# Autodesk Inventor assembly: slozene
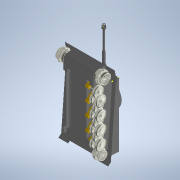
[picture p0: Inventor's stored thumbnail of the model, 180x180]
Saved by Autodesk Inventor 2022 (Build 260153000, 153)
## iProperties
Created: 2022-11-15
Part Number: slozene
Document SubType Name: Assembly
Designer: matys
Author: matys
## Documents named in this file (24)
- C:\Users\matys\Desktop\Práce4tak\Inventor\novy tank\model\slozene.iam
- C:\Users\matys\Desktop\Práce4tak\Inventor\novy tank\model\dolni-cast.ipt
- C:\Users\matys\Desktop\Práce4tak\Inventor\model_v1\motor.ipt
- C:\Users\matys\Desktop\Práce4tak\Inventor\novy tank\ozubene-kolo.ipt
- C:\Users\matys\Desktop\Práce4tak\Inventor\mechanismus_odpruzeni\pist.ipt
- C:\Users\matys\Desktop\Práce4tak\Inventor\mechanismus_odpruzeni\pist-dolni.ipt
- C:\Users\matys\Desktop\Práce4tak\Inventor\mechanismus_odpruzeni\pist-zatka.ipt
- C:\Users\matys\Desktop\Práce4tak\Inventor\mechanismus_odpruzeni\mid.ipt
- C:\Users\matys\Desktop\Práce4tak\Inventor\novy tank\tycinka.ipt
- C:\Users\matys\Desktop\Práce4tak\Inventor\novy tank\tycinka_12mm.ipt
- C:\Users\matys\Desktop\Práce4tak\Inventor\novy tank\spring.ipt
- C:\Users\matys\Desktop\Práce4tak\Inventor\novy tank\tycinka_dlouha.ipt
- C:\Users\matys\Desktop\Práce4tak\Inventor\novy tank\kolo_mensi.ipt
- C:\Users\matys\Desktop\Práce4tak\Inventor\novy tank\sroub.ipt
- C:\Users\matys\Desktop\Práce4tak\Inventor\novy tank\tycinka_kratsi.ipt
- C:\Users\matys\Desktop\Práce4tak\Inventor\novy tank\kolo_vetsi.ipt
- C:\Users\matys\Desktop\Práce4tak\Inventor\novy tank\ozubene-kolo_mini.ipt
- C:\Users\matys\Desktop\Práce4tak\Inventor\baterka.ipt
- C:\Users\matys\Desktop\Práce4tak\Inventor\model_v1\L298N.ipt
- C:\Users\matys\Desktop\Práce4tak\Inventor\novy tank\model\horni-cast.ipt
- C:\Users\matys\Desktop\Práce4tak\Inventor\novy tank\model\vez.ipt
- C:\Users\matys\Desktop\Práce4tak\Inventor\novy tank\model\vez-rotate.ipt
- C:\Users\matys\Desktop\Práce4tak\Inventor\novy tank\model\vez-delo-plate.ipt
- C:\Users\matys\Desktop\Práce4tak\Inventor\novy tank\model\delo.ipt
## Components (103 placed, 23 different names)
1. dolni-cast:1 — Mate:1, Mate:2, Mate:3, Mate:4, Mate:24, Mate:25, Mate:26, Mate:27, Mate:28, Mate:29, Mate:38, Mate:39, Mate:40, Mate:41, Mate:48, Mate:50, Mate:58, Mate:59, Mate:60, Mate:61, Mate:70, Mate:81, Mate:88, Mate:89, Mate:90, Mate:91, Mate:92, Mate:93, Mate:94, Mate:95, Mate:96, Mate:97, Mate:98, Mate:99, Mate:100, Mate:101, Mate:102, Mate:103, Mate:104, Mate:105, Mate:106, Mate:107, Mate:127, Mate:129, Mate:131, Mate:133, Mate:135, Mate:137, Mate:139, Mate:141, Mate:143, Mate:145, Mate:196, Mate:204
2. motor:1 — Mate:3, Mate:4, Mate:204, Mate:205
3. motor:2 — Mate:1, Mate:2, Mate:5, Mate:6
4. ozubene-kolo:1 — Mate:5, Mate:6
5. pist:1 — Mate:7, Mate:8, Mate:9, Mate:10, Mate:22, Mate:23, Mate:29
6. pist-dolni:1 — Mate:10, Mate:11, Mate:21
7. pist-zatka:1 — Mate:7, Mate:8, Mate:11
8. mid:1 — Mate:15, Mate:19, Mate:20, Mate:26, Mate:30, Mate:31
9. tycinka:1 — Mate:15, Mate:24, Mate:25
10. tycinka:2 — Mate:9, Mate:27, Mate:28
11. tycinka_12mm:1 — Mate:19, Mate:20, Mate:21
12. spring:1 — Mate:22, Mate:23
13. kolo_mensi:2 — Mate:32, Mate:35
14. sroub:1 — Mate:33, Mate:34, Mate:35
15. tycinka_kratsi:1 — Mate:30, Mate:31, Mate:32, Mate:33, Mate:34
16. tycinka_kratsi:2 — Mate:52, Mate:53, Mate:54, Mate:55, Mate:56
17. sroub:2 — Mate:54, Mate:55, Mate:57
18. spring:2 — Mate:44, Mate:45
19. tycinka_12mm:2 — Mate:42, Mate:43, Mate:51
20. tycinka:3 — Mate:40, Mate:41, Mate:49
21. tycinka:4 — Mate:38, Mate:39, Mate:47
22. mid:2 — Mate:42, Mate:43, Mate:47, Mate:48, Mate:52, Mate:53
23. pist:2 — Mate:36, Mate:37, Mate:44, Mate:45, Mate:46, Mate:49, Mate:50
24. pist-dolni:2 — Mate:46, Mate:51
25. pist-zatka:2 — Mate:36, Mate:37
26. kolo_mensi:3 — Mate:56, Mate:57
27. tycinka:5 — Mate:60, Mate:61, Mate:69
28. tycinka:6 — Mate:58, Mate:59, Mate:80
29. tycinka_12mm:3 — Mate:73, Mate:82, Mate:83
30. kolo_vetsi:1 — Mate:76, Mate:79
31. tycinka_dlouha:1 — Mate:76, Mate:77, Mate:78, Mate:84, Mate:85
32. pist:3 — Mate:62, Mate:65, Mate:68, Mate:69, Mate:70
33. pist-dolni:3 — Mate:66, Mate:73
34. pist-zatka:3 — Mate:67, Mate:68
35. spring:3 — Mate:62, Mate:65, Mate:66, Mate:67
36. sroub:3 — Mate:77, Mate:78, Mate:79
37. mid:3 — Mate:80, Mate:81, Mate:82, Mate:83, Mate:84, Mate:85
38. tycinka:7 — Mate:101, Mate:105, Mate:140
39. tycinka:8 — Mate:100, Mate:104, Mate:134
40. tycinka:9 — Mate:98, Mate:99, Mate:130
41. tycinka:10 — Mate:92, Mate:93, Mate:144
42. tycinka:11 — Mate:102, Mate:107, Mate:142
43. tycinka:12 — Mate:96, Mate:97, Mate:138
44. tycinka:13 — Mate:94, Mate:95, Mate:128
45. tycinka:14 — Mate:90, Mate:91, Mate:126
46. tycinka:15 — Mate:103, Mate:106, Mate:132
47. tycinka:16 — Mate:88, Mate:89, Mate:136
48. tycinka_12mm:4 — Mate:116, Mate:117, Mate:157
49. tycinka_12mm:5 — Mate:109, Mate:112, Mate:164
50. tycinka_12mm:6 — Mate:114, Mate:115, Mate:163
51. tycinka_12mm:7 — Mate:110, Mate:111, Mate:159
52. tycinka_12mm:8 — Mate:108, Mate:113, Mate:165
53. spring:4 — Mate:151, Mate:155
54. spring:5 — Mate:150, Mate:154
55. spring:6 — Mate:149, Mate:153
56. spring:7 — Mate:148, Mate:152
57. spring:8 — Mate:146, Mate:147
58. tycinka_dlouha:2 — Mate:166, Mate:169, Mate:192, Mate:193
59. tycinka_dlouha:3 — Mate:167, Mate:170, Mate:191, Mate:194
60. tycinka_dlouha:4 — Mate:168, Mate:171, Mate:190, Mate:195
61. tycinka_kratsi:3 — Mate:172, Mate:174, Mate:180, Mate:181
62. tycinka_kratsi:4 — Mate:173, Mate:175, Mate:182, Mate:183
63. sroub:4 — Mate:184, Mate:187, Mate:191, Mate:194
64. sroub:5 — Mate:185, Mate:189, Mate:190, Mate:195
65. sroub:6 — Mate:186, Mate:188, Mate:192, Mate:193
66. sroub:7 — Mate:176, Mate:178, Mate:180, Mate:181
67. sroub:8 — Mate:177, Mate:179, Mate:182, Mate:183
68. kolo_vetsi:2 — Mate:184, Mate:187
69. kolo_vetsi:3 — Mate:186, Mate:188
70. kolo_vetsi:4 — Mate:185, Mate:189
71. kolo_mensi:4 — Mate:177, Mate:179
72. kolo_mensi:5 — Mate:176, Mate:178
73. mid:4 — Mate:114, Mate:115, Mate:142, Mate:143, Mate:172, Mate:174
74. mid:5 — Mate:116, Mate:117, Mate:136, Mate:137, Mate:166, Mate:169
75. mid:6 — Mate:110, Mate:111, Mate:144, Mate:145, Mate:167, Mate:170
76. mid:7 — Mate:109, Mate:112, Mate:140, Mate:141, Mate:173, Mate:175
77. mid:8 — Mate:108, Mate:113, Mate:138, Mate:139, Mate:168, Mate:171
78. pist:4 — Mate:86, Mate:87, Mate:134, Mate:135, Mate:150, Mate:154, Mate:162
79. pist:5 — Mate:118, Mate:122, Mate:132, Mate:133, Mate:148, Mate:152, Mate:160
80. pist:6 — Mate:119, Mate:123, Mate:130, Mate:131, Mate:151, Mate:155, Mate:161
81. pist:7 — Mate:120, Mate:124, Mate:128, Mate:129, Mate:149, Mate:153, Mate:158
82. pist:8 — Mate:121, Mate:125, Mate:126, Mate:127, Mate:146, Mate:147, Mate:156
83. pist-dolni:4 — Mate:161, Mate:165
84. pist-dolni:5 — Mate:158, Mate:159
85. pist-dolni:6 — Mate:160, Mate:163
86. pist-dolni:7 — Mate:162, Mate:164
87. pist-dolni:8 — Mate:156, Mate:157
88. pist-zatka:4 — Mate:118, Mate:122
89. pist-zatka:5 — Mate:119, Mate:123
90. pist-zatka:6 — Mate:120, Mate:124
91. pist-zatka:7 — Mate:121, Mate:125
92. pist-zatka:8 — Mate:86, Mate:87
93. tycinka_kratsi:5 — Mate:196, Mate:197, Mate:198
94. ozubene-kolo_mini:1 — Mate:197, Mate:199
95. sroub:9 — Mate:198, Mate:199
96. baterka:1
97. L298N:1
98. horni-cast:1 — Mate:202
99. vez:1 — Mate:200, Mate:201, Mate:203
100. vez-rotate:1 — Mate:200, Mate:201, Mate:202
101. vez-delo-plate:1 — Mate:203
102. ozubene-kolo:2 — Mate:205
103. delo:1
## Relationships (193: Mate 193)
- Mate:1: dolni-cast:1 ↔ motor:2
- Mate:2: dolni-cast:1 ↔ motor:2
- Mate:3: dolni-cast:1 ↔ motor:1
- Mate:4: dolni-cast:1 ↔ motor:1
- Mate:5: motor:2 ↔ ozubene-kolo:1
- Mate:6: motor:2 ↔ ozubene-kolo:1
- Mate:7: pist:1 ↔ pist-zatka:1
- Mate:8: pist:1 ↔ pist-zatka:1
- Mate:9: pist:1 ↔ tycinka:2
- Mate:10: pist:1 ↔ pist-dolni:1
- Mate:11: pist-dolni:1 ↔ pist-zatka:1
- Mate:15: mid:1 ↔ tycinka:1
- Mate:19: mid:1 ↔ tycinka_12mm:1
- Mate:20: mid:1 ↔ tycinka_12mm:1
- Mate:21: pist-dolni:1 ↔ tycinka_12mm:1
- Mate:22: pist:1 ↔ spring:1
- Mate:23: pist:1 ↔ spring:1
- Mate:24: dolni-cast:1 ↔ tycinka:1
- Mate:25: dolni-cast:1 ↔ tycinka:1
- Mate:26: dolni-cast:1 ↔ mid:1
- Mate:27: dolni-cast:1 ↔ tycinka:2
- Mate:28: dolni-cast:1 ↔ tycinka:2
- Mate:29: dolni-cast:1 ↔ pist:1
- Mate:30: mid:1 ↔ tycinka_kratsi:1
- Mate:31: mid:1 ↔ tycinka_kratsi:1
- Mate:32: kolo_mensi:2 ↔ tycinka_kratsi:1
- Mate:33: sroub:1 ↔ tycinka_kratsi:1
- Mate:34: sroub:1 ↔ tycinka_kratsi:1
- Mate:35: kolo_mensi:2 ↔ sroub:1
- Mate:36: pist:2 ↔ pist-zatka:2
- Mate:37: pist:2 ↔ pist-zatka:2
- Mate:38: dolni-cast:1 ↔ tycinka:4
- Mate:39: dolni-cast:1 ↔ tycinka:4
- Mate:40: dolni-cast:1 ↔ tycinka:3
- Mate:41: dolni-cast:1 ↔ tycinka:3
- Mate:42: tycinka_12mm:2 ↔ mid:2
- Mate:43: tycinka_12mm:2 ↔ mid:2
- Mate:44: spring:2 ↔ pist:2
- Mate:45: spring:2 ↔ pist:2
- Mate:46: pist:2 ↔ pist-dolni:2
- Mate:47: tycinka:4 ↔ mid:2
- Mate:48: dolni-cast:1 ↔ mid:2
- Mate:49: tycinka:3 ↔ pist:2
- Mate:50: dolni-cast:1 ↔ pist:2
- Mate:51: tycinka_12mm:2 ↔ pist-dolni:2
- Mate:52: tycinka_kratsi:2 ↔ mid:2
- Mate:53: tycinka_kratsi:2 ↔ mid:2
- Mate:54: tycinka_kratsi:2 ↔ sroub:2
- Mate:55: tycinka_kratsi:2 ↔ sroub:2
- Mate:56: tycinka_kratsi:2 ↔ kolo_mensi:3
- Mate:57: sroub:2 ↔ kolo_mensi:3
- Mate:58: dolni-cast:1 ↔ tycinka:6
- Mate:59: dolni-cast:1 ↔ tycinka:6
- Mate:60: dolni-cast:1 ↔ tycinka:5
- Mate:61: dolni-cast:1 ↔ tycinka:5
- Mate:62: pist:3 ↔ spring:3
- Mate:65: pist:3 ↔ spring:3
- Mate:66: pist-dolni:3 ↔ spring:3
- Mate:67: pist-zatka:3 ↔ spring:3
- Mate:68: pist:3 ↔ pist-zatka:3
- Mate:69: tycinka:5 ↔ pist:3
- Mate:70: dolni-cast:1 ↔ pist:3
- Mate:73: tycinka_12mm:3 ↔ pist-dolni:3
- Mate:76: kolo_vetsi:1 ↔ tycinka_dlouha:1
- Mate:77: tycinka_dlouha:1 ↔ sroub:3
- Mate:78: tycinka_dlouha:1 ↔ sroub:3
- Mate:79: kolo_vetsi:1 ↔ sroub:3
- Mate:80: tycinka:6 ↔ mid:3
- Mate:81: dolni-cast:1 ↔ mid:3
- Mate:82: tycinka_12mm:3 ↔ mid:3
- Mate:83: tycinka_12mm:3 ↔ mid:3
- Mate:84: tycinka_dlouha:1 ↔ mid:3
- Mate:85: tycinka_dlouha:1 ↔ mid:3
- Mate:86: pist:4 ↔ pist-zatka:8
- Mate:87: pist:4 ↔ pist-zatka:8
- Mate:88: dolni-cast:1 ↔ tycinka:16
- Mate:89: dolni-cast:1 ↔ tycinka:16
- Mate:90: dolni-cast:1 ↔ tycinka:14
- Mate:91: dolni-cast:1 ↔ tycinka:14
- Mate:92: dolni-cast:1 ↔ tycinka:10
- Mate:93: dolni-cast:1 ↔ tycinka:10
- Mate:94: dolni-cast:1 ↔ tycinka:13
- Mate:95: dolni-cast:1 ↔ tycinka:13
- Mate:96: dolni-cast:1 ↔ tycinka:12
- Mate:97: dolni-cast:1 ↔ tycinka:12
- Mate:98: dolni-cast:1 ↔ tycinka:9
- Mate:99: dolni-cast:1 ↔ tycinka:9
- Mate:100: dolni-cast:1 ↔ tycinka:8
- Mate:101: dolni-cast:1 ↔ tycinka:7
- Mate:102: dolni-cast:1 ↔ tycinka:11
- Mate:103: dolni-cast:1 ↔ tycinka:15
- Mate:104: dolni-cast:1 ↔ tycinka:8
- Mate:105: dolni-cast:1 ↔ tycinka:7
- Mate:106: dolni-cast:1 ↔ tycinka:15
- Mate:107: dolni-cast:1 ↔ tycinka:11
- Mate:108: tycinka_12mm:8 ↔ mid:8
- Mate:109: tycinka_12mm:5 ↔ mid:7
- Mate:110: tycinka_12mm:7 ↔ mid:6
- Mate:111: tycinka_12mm:7 ↔ mid:6
- Mate:112: tycinka_12mm:5 ↔ mid:7
- Mate:113: tycinka_12mm:8 ↔ mid:8
- Mate:114: tycinka_12mm:6 ↔ mid:4
- Mate:115: tycinka_12mm:6 ↔ mid:4
- Mate:116: tycinka_12mm:4 ↔ mid:5
- Mate:117: tycinka_12mm:4 ↔ mid:5
- Mate:118: pist:5 ↔ pist-zatka:4
- Mate:119: pist:6 ↔ pist-zatka:5
- Mate:120: pist:7 ↔ pist-zatka:6
- Mate:121: pist:8 ↔ pist-zatka:7
- Mate:122: pist:5 ↔ pist-zatka:4
- Mate:123: pist:6 ↔ pist-zatka:5
- Mate:124: pist:7 ↔ pist-zatka:6
- Mate:125: pist:8 ↔ pist-zatka:7
- Mate:126: tycinka:14 ↔ pist:8
- Mate:127: dolni-cast:1 ↔ pist:8
- Mate:128: tycinka:13 ↔ pist:7
- Mate:129: dolni-cast:1 ↔ pist:7
- Mate:130: tycinka:9 ↔ pist:6
- Mate:131: dolni-cast:1 ↔ pist:6
- Mate:132: tycinka:15 ↔ pist:5
- Mate:133: dolni-cast:1 ↔ pist:5
- Mate:134: tycinka:8 ↔ pist:4
- Mate:135: dolni-cast:1 ↔ pist:4
- Mate:136: tycinka:16 ↔ mid:5
- Mate:137: dolni-cast:1 ↔ mid:5
- Mate:138: tycinka:12 ↔ mid:8
- Mate:139: dolni-cast:1 ↔ mid:8
- Mate:140: tycinka:7 ↔ mid:7
- Mate:141: dolni-cast:1 ↔ mid:7
- Mate:142: tycinka:11 ↔ mid:4
- Mate:143: dolni-cast:1 ↔ mid:4
- Mate:144: tycinka:10 ↔ mid:6
- Mate:145: dolni-cast:1 ↔ mid:6
- Mate:146: spring:8 ↔ pist:8
- Mate:147: spring:8 ↔ pist:8
- Mate:148: spring:7 ↔ pist:5
- Mate:149: spring:6 ↔ pist:7
- Mate:150: spring:5 ↔ pist:4
- Mate:151: spring:4 ↔ pist:6
- Mate:152: spring:7 ↔ pist:5
- Mate:153: spring:6 ↔ pist:7
- Mate:154: spring:5 ↔ pist:4
- Mate:155: spring:4 ↔ pist:6
- Mate:156: pist:8 ↔ pist-dolni:8
- Mate:157: tycinka_12mm:4 ↔ pist-dolni:8
- Mate:158: pist:7 ↔ pist-dolni:5
- Mate:159: tycinka_12mm:7 ↔ pist-dolni:5
- Mate:160: pist:5 ↔ pist-dolni:6
- Mate:161: pist:6 ↔ pist-dolni:4
- Mate:162: pist:4 ↔ pist-dolni:7
- Mate:163: tycinka_12mm:6 ↔ pist-dolni:6
- Mate:164: tycinka_12mm:5 ↔ pist-dolni:7
- Mate:165: tycinka_12mm:8 ↔ pist-dolni:4
- Mate:166: tycinka_dlouha:2 ↔ mid:5
- Mate:167: tycinka_dlouha:3 ↔ mid:6
- Mate:168: tycinka_dlouha:4 ↔ mid:8
- Mate:169: tycinka_dlouha:2 ↔ mid:5
- Mate:170: tycinka_dlouha:3 ↔ mid:6
- Mate:171: tycinka_dlouha:4 ↔ mid:8
- Mate:172: tycinka_kratsi:3 ↔ mid:4
- Mate:173: tycinka_kratsi:4 ↔ mid:7
- Mate:174: tycinka_kratsi:3 ↔ mid:4
- Mate:175: tycinka_kratsi:4 ↔ mid:7
- Mate:176: sroub:7 ↔ kolo_mensi:5
- Mate:177: sroub:8 ↔ kolo_mensi:4
- Mate:178: sroub:7 ↔ kolo_mensi:5
- Mate:179: sroub:8 ↔ kolo_mensi:4
- Mate:180: tycinka_kratsi:3 ↔ sroub:7
- Mate:181: tycinka_kratsi:3 ↔ sroub:7
- Mate:182: tycinka_kratsi:4 ↔ sroub:8
- Mate:183: tycinka_kratsi:4 ↔ sroub:8
- Mate:184: sroub:4 ↔ kolo_vetsi:2
- Mate:185: sroub:5 ↔ kolo_vetsi:4
- Mate:186: sroub:6 ↔ kolo_vetsi:3
- Mate:187: sroub:4 ↔ kolo_vetsi:2
- Mate:188: sroub:6 ↔ kolo_vetsi:3
- Mate:189: sroub:5 ↔ kolo_vetsi:4
- Mate:190: tycinka_dlouha:4 ↔ sroub:5
- Mate:191: tycinka_dlouha:3 ↔ sroub:4
- Mate:192: tycinka_dlouha:2 ↔ sroub:6
- Mate:193: tycinka_dlouha:2 ↔ sroub:6
- Mate:194: tycinka_dlouha:3 ↔ sroub:4
- Mate:195: tycinka_dlouha:4 ↔ sroub:5
- Mate:196: dolni-cast:1 ↔ tycinka_kratsi:5
- Mate:197: tycinka_kratsi:5 ↔ ozubene-kolo_mini:1
- Mate:198: tycinka_kratsi:5 ↔ sroub:9
- Mate:199: ozubene-kolo_mini:1 ↔ sroub:9
- Mate:200: vez:1 ↔ vez-rotate:1
- Mate:201: vez:1 ↔ vez-rotate:1
- Mate:202: horni-cast:1 ↔ vez-rotate:1
- Mate:203: vez:1 ↔ vez-delo-plate:1
- Mate:204: dolni-cast:1 ↔ motor:1
- Mate:205: motor:1 ↔ ozubene-kolo:2
